# Autodesk Inventor assembly: Assembly1
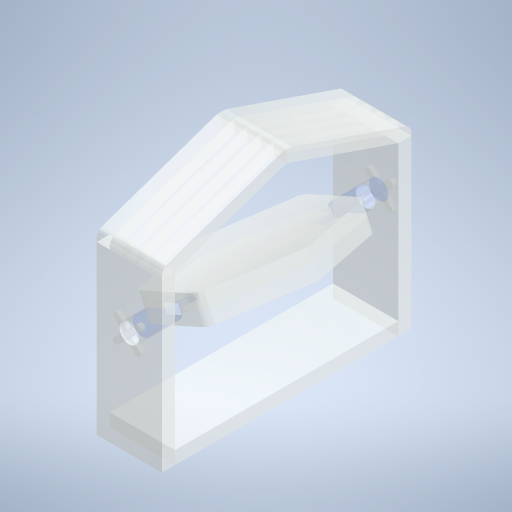
[picture p0: Inventor's stored thumbnail of the model, 512x512]
Saved by Autodesk Inventor 2023.1 (Build 271208000, 208)
## iProperties
Created: 2022-10-28
Part Number: Assembly1
Document SubType Name: Assembly
Designer: jshin23
Author: jshin23
## Documents named in this file (7)
- C:\Users\jshin23\Desktop\Kids Toy\Assembly1.iam
- C:\Users\jshin23\Desktop\Kids Toy\Part1 x 2.ipt
- C:\Users\jshin23\Desktop\Kids Toy\Part2 x 1.ipt
- C:\Users\jshin23\Desktop\Kids Toy\Part3 x 2.ipt
- C:\Users\jshin23\Desktop\Kids Toy\3DPart6 x 2.ipt
- C:\Users\jshin23\Desktop\Kids Toy\Part4 x 12.ipt
- C:\Users\jshin23\Desktop\Kids Toy\3DPart7 x 2.ipt
## Components (19 placed, 6 different names)
1. Part2 x 1:1 — Mate:1, Flush:1, Flush:2, Mate:2, Flush:3, Flush:4
2. Part3 x 2:1 — Mate:1, Flush:1, Flush:2, Mate:11, Flush:7
3. Part3 x 2:2 — Mate:2, Flush:3, Flush:4, Mate:13, Flush:10, Flush:11
4. 3DPart6 x 2:1 — Mate:7, Mate:8, Mate:9, Mate:23
5. 3DPart6 x 2:2 — Mate:4, Mate:5, Mate:6, Mate:11, Flush:7, Mate:24
6. Part1 x 2:1 — Mate:3, Flush:5, Flush:6, Mate:4, Mate:5, Mate:7, Mate:8
7. Part1 x 2:2 — Mate:3, Flush:5, Flush:6, Mate:6, Mate:9
8. Part4 x 12:1 — Flush:8, Flush:9, Mate:14, Flush:27
9. Part4 x 12:2 — Mate:15, Flush:14, Flush:15, Flush:24, Flush:25, Flush:27
10. Part4 x 12:3 — Mate:15, Mate:16, Flush:13, Flush:15, Flush:16
11. Part4 x 12:4 — Mate:17, Flush:12, Flush:17
12. Part4 x 12:5 — Mate:18, Flush:18, Flush:21
13. Part4 x 12:6 — Mate:18, Mate:19, Flush:18, Flush:19, Flush:21, Flush:23
14. Part4 x 12:7 — Mate:19, Mate:20, Flush:19, Flush:20, Flush:22, Flush:23, Mate:21
15. Part4 x 12:8 — Mate:20, Flush:20, Flush:22, Flush:24, Flush:25, Mate:22, Flush:26
16. Part4 x 12:9 — Flush:8, Flush:9, Mate:13, Flush:10, Mate:14, Flush:11, Mate:22, Flush:26
17. Part4 x 12:10 — Mate:16, Mate:17, Flush:12, Flush:13, Flush:14, Flush:16, Flush:17, Mate:21
18. 3DPart7 x 2:1 — Mate:24
19. 3DPart7 x 2:2 — Mate:23
## Relationships (49: Flush 27, Mate 22)
- Mate:1: Part2 x 1:1 ↔ Part3 x 2:1
- Flush:1: Part2 x 1:1 ↔ Part3 x 2:1
- Flush:2: Part2 x 1:1 ↔ Part3 x 2:1
- Mate:2: Part2 x 1:1 ↔ Part3 x 2:2
- Flush:3: Part2 x 1:1 ↔ Part3 x 2:2
- Flush:4: Part2 x 1:1 ↔ Part3 x 2:2
- Mate:3: Part1 x 2:1 ↔ Part1 x 2:2
- Flush:5: Part1 x 2:1 ↔ Part1 x 2:2
- Flush:6: Part1 x 2:1 ↔ Part1 x 2:2
- Mate:4: 3DPart6 x 2:2 ↔ Part1 x 2:1
- Mate:5: 3DPart6 x 2:2 ↔ Part1 x 2:1
- Mate:6: 3DPart6 x 2:2 ↔ Part1 x 2:2
- Mate:7: 3DPart6 x 2:1 ↔ Part1 x 2:1
- Mate:8: 3DPart6 x 2:1 ↔ Part1 x 2:1
- Mate:9: 3DPart6 x 2:1 ↔ Part1 x 2:2
- Mate:11: Part3 x 2:1 ↔ 3DPart6 x 2:2
- Flush:7: Part3 x 2:1 ↔ 3DPart6 x 2:2
- Flush:8: Part4 x 12:1 ↔ Part4 x 12:9
- Flush:9: Part4 x 12:1 ↔ Part4 x 12:9
- Mate:13: Part3 x 2:2 ↔ Part4 x 12:9
- Flush:10: Part3 x 2:2 ↔ Part4 x 12:9
- Mate:14: Part4 x 12:1 ↔ Part4 x 12:9
- Flush:11: Part3 x 2:2 ↔ Part4 x 12:9
- Mate:15: Part4 x 12:2 ↔ Part4 x 12:3
- Mate:16: Part4 x 12:3 ↔ Part4 x 12:10
- Mate:17: Part4 x 12:4 ↔ Part4 x 12:10
- Flush:12: Part4 x 12:4 ↔ Part4 x 12:10
- Flush:13: Part4 x 12:3 ↔ Part4 x 12:10
- Flush:14: Part4 x 12:2 ↔ Part4 x 12:10
- Flush:15: Part4 x 12:2 ↔ Part4 x 12:3
- Flush:16: Part4 x 12:3 ↔ Part4 x 12:10
- Flush:17: Part4 x 12:4 ↔ Part4 x 12:10
- Mate:18: Part4 x 12:5 ↔ Part4 x 12:6
- Mate:19: Part4 x 12:6 ↔ Part4 x 12:7
- Mate:20: Part4 x 12:7 ↔ Part4 x 12:8
- Flush:18: Part4 x 12:5 ↔ Part4 x 12:6
- Flush:19: Part4 x 12:6 ↔ Part4 x 12:7
- Flush:20: Part4 x 12:7 ↔ Part4 x 12:8
- Flush:21: Part4 x 12:5 ↔ Part4 x 12:6
- Flush:22: Part4 x 12:7 ↔ Part4 x 12:8
- Flush:23: Part4 x 12:6 ↔ Part4 x 12:7
- Mate:21: Part4 x 12:7 ↔ Part4 x 12:10
- Flush:24: Part4 x 12:2 ↔ Part4 x 12:8
- Flush:25: Part4 x 12:2 ↔ Part4 x 12:8
- Mate:22: Part4 x 12:8 ↔ Part4 x 12:9
- Flush:26: Part4 x 12:8 ↔ Part4 x 12:9
- Flush:27: Part4 x 12:1 ↔ Part4 x 12:2
- Mate:23: 3DPart6 x 2:1 ↔ 3DPart7 x 2:2
- Mate:24: 3DPart6 x 2:2 ↔ 3DPart7 x 2:1
